# Autodesk Inventor assembly: Assembly 1
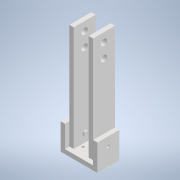
[picture p0: Inventor's stored thumbnail of the model, 180x180]
Saved by Autodesk Inventor 2022 (Build 260153000, 153)
## iProperties
Created: 2022-06-16
Part Number: Assembly 1
Document SubType Name: Assembly
Designer: chait
Author: chait
## Documents named in this file (4)
- C:\Users\chait\Documents\Assembly 1.iam
- C:\Users\chait\Documents\clamp.ipt
- C:\Users\chait\Documents\Stationary arm 2.ipt
- C:\Users\chait\Documents\Screw 3mm.ipt
## Components (5 placed, 3 different names)
1. clamp:1 — Insert:1, Insert:3
2. Stationary arm 2:1 — Insert:2
3. Stationary arm 2:2 — Insert:1
4. Screw 3mm:1
5. Screw 3mm:2 — Insert:2, Insert:3
## Relationships (3: Insert 3)
- Insert:1: clamp:1 ↔ Stationary arm 2:2
- Insert:2: Stationary arm 2:1 ↔ Screw 3mm:2
- Insert:3: clamp:1 ↔ Screw 3mm:2
